# Autodesk Inventor assembly: mobile_robot
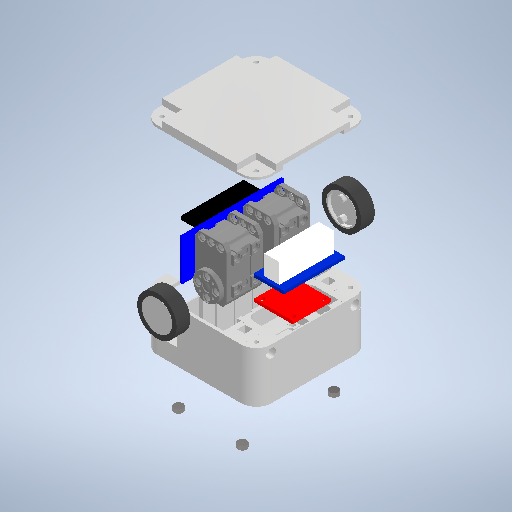
[picture p0: Inventor's stored thumbnail of the model, 512x512]
Saved by Autodesk Inventor 2025 (Build 290162000, 162)
## iProperties
Created: 2025-10-18
Part Number: mobile_robot
Document SubType Name: Assembly
Designer: sooo1
Author: sooo1
## Documents named in this file (13)
- C:\Users\sooo1\Downloads\final-20260216T060151Z-1-001\final\mobile_robot\mobile_robot_disassemble.iam
- C:\Users\sooo1\Downloads\final-20260216T060151Z-1-001\final\mobile_robot\enclosure.ipt
- C:\Users\sooo1\Downloads\final-20260216T060151Z-1-001\final\mobile_robot\XL-320.ipt
- C:\Users\sooo1\Downloads\final-20260216T060151Z-1-001\final\mobile_robot\wheel.ipt
- C:\Users\sooo1\Downloads\final-20260216T060151Z-1-001\final\mobile_robot\tire_20-26.ipt
- C:\Users\sooo1\Downloads\final-20260216T060151Z-1-001\final\mobile_robot\odometry.ipt
- C:\Users\sooo1\Downloads\final-20260216T060151Z-1-001\final\mobile_robot\i2chub.ipt
- C:\Users\sooo1\Downloads\final-20260216T060151Z-1-001\final\mobile_robot\housing_motor.ipt
- C:\Users\sooo1\Downloads\final-20260216T060151Z-1-001\final\mobile_robot\lid.ipt
- C:\Users\sooo1\Downloads\final-20260216T060151Z-1-001\final\mobile_robot\opencm9.04.ipt
- C:\Users\sooo1\Downloads\final-20260216T060151Z-1-001\final\mobile_robot\plate_ball.ipt
- C:\Users\sooo1\Downloads\final-20260216T060151Z-1-001\final\mobile_robot\ball.ipt
- C:\Users\sooo1\Downloads\final-20260216T060151Z-1-001\final\mobile_robot\neodymiummagnet_Φ6.ipt
## Components (20 placed, 12 different names)
1. enclosure:1 — メイト:1, フラッシュ:3, メイト:2, メイト:3, メイト:4, メイト:5, メイト:8, メイト:9, メイト:10, メイト:11, メイト:14, メイト:15, メイト:18, メイト:19, メイト:20, メイト:24, メイト:25, メイト:28, メイト:29, メイト:34
2. XL-320:1 — メイト:30, メイト:31, メイト:32, メイト:33, メイト:34
3. XL-320:2 — メイト:21, メイト:22, メイト:32, メイト:33
4. wheel:1 — メイト:26, メイト:27, メイト:30, メイト:31
5. wheel:2 — メイト:21, メイト:22, メイト:23, フラッシュ:11
6. tire_20-26:1 — メイト:26, メイト:27
7. tire_20-26:2 — メイト:23, フラッシュ:11
8. odometry:1 — メイト:28, メイト:29
9. i2chub:1
10. housing_motor:1 — メイト:3, メイト:4, メイト:5
11. lid:1 — フラッシュ:4, メイト:2
12. opencm9.04:1 — メイト:24, メイト:25
13. plate_ball:1 — メイト:12, メイト:13, フラッシュ:8, メイト:14, メイト:15, フラッシュ:10, メイト:20
14. ball:1 — メイト:12, メイト:13, フラッシュ:8
15. neodymiummagnet_Φ6:1 — メイト:8, フラッシュ:6, フラッシュ:7
16. neodymiummagnet_Φ6:2 — メイト:9, フラッシュ:7
17. neodymiummagnet_Φ6:3 — メイト:11, フラッシュ:5
18. neodymiummagnet_Φ6:4 — メイト:10, フラッシュ:5, フラッシュ:6
19. plate_ball:2 — メイト:18, メイト:19, フラッシュ:10
20. ball:2
## Relationships (41: Mate 32, Flush 9)
- メイト:1 [Mate]: enclosure:1
- フラッシュ:3 [Flush]: enclosure:1
- フラッシュ:4 [Flush]: lid:1
- メイト:2 [Mate]: enclosure:1 ↔ lid:1
- メイト:3 [Mate]: enclosure:1 ↔ housing_motor:1
- メイト:4 [Mate]: enclosure:1 ↔ housing_motor:1
- メイト:5 [Mate]: enclosure:1 ↔ housing_motor:1
- メイト:8 [Mate]: enclosure:1 ↔ neodymiummagnet_Φ6:1
- メイト:9 [Mate]: enclosure:1 ↔ neodymiummagnet_Φ6:2
- メイト:10 [Mate]: enclosure:1 ↔ neodymiummagnet_Φ6:4
- メイト:11 [Mate]: enclosure:1 ↔ neodymiummagnet_Φ6:3
- フラッシュ:5 [Flush]: neodymiummagnet_Φ6:3 ↔ neodymiummagnet_Φ6:4
- フラッシュ:6 [Flush]: neodymiummagnet_Φ6:1 ↔ neodymiummagnet_Φ6:4
- フラッシュ:7 [Flush]: neodymiummagnet_Φ6:1 ↔ neodymiummagnet_Φ6:2
- メイト:12 [Mate]: plate_ball:1 ↔ ball:1
- メイト:13 [Mate]: plate_ball:1 ↔ ball:1
- フラッシュ:8 [Flush]: plate_ball:1 ↔ ball:1
- メイト:14 [Mate]: enclosure:1 ↔ plate_ball:1
- メイト:15 [Mate]: enclosure:1 ↔ plate_ball:1
- [Mate]: plate_ball:2 ↔ ball:2
- [Mate]: plate_ball:2 ↔ ball:2
- [Flush]: plate_ball:2 ↔ ball:2
- メイト:18 [Mate]: enclosure:1 ↔ plate_ball:2
- メイト:19 [Mate]: enclosure:1 ↔ plate_ball:2
- フラッシュ:10 [Flush]: plate_ball:1 ↔ plate_ball:2
- メイト:20 [Mate]: enclosure:1 ↔ plate_ball:1
- メイト:21 [Mate]: XL-320:2 ↔ wheel:2
- メイト:22 [Mate]: XL-320:2 ↔ wheel:2
- メイト:23 [Mate]: wheel:2 ↔ tire_20-26:2
- フラッシュ:11 [Flush]: wheel:2 ↔ tire_20-26:2
- メイト:24 [Mate]: enclosure:1 ↔ opencm9.04:1
- メイト:25 [Mate]: enclosure:1 ↔ opencm9.04:1
- メイト:26 [Mate]: wheel:1 ↔ tire_20-26:1
- メイト:27 [Mate]: wheel:1 ↔ tire_20-26:1
- メイト:28 [Mate]: enclosure:1 ↔ odometry:1
- メイト:29 [Mate]: enclosure:1 ↔ odometry:1
- メイト:30 [Mate]: XL-320:1 ↔ wheel:1
- メイト:31 [Mate]: XL-320:1 ↔ wheel:1
- メイト:32 [Mate]: XL-320:1 ↔ XL-320:2
- メイト:33 [Mate]: XL-320:1 ↔ XL-320:2
- メイト:34 [Mate]: enclosure:1 ↔ XL-320:1
## Named parameters: d179_d174 = 0 mm, d180_d175 = 0 mm, d181_d176 = 0 mm
